# Autodesk Inventor assembly: Arm_v2
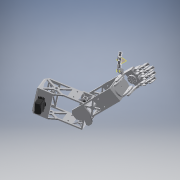
[picture p0: Inventor's stored thumbnail of the model, 180x180]
Saved by Autodesk Inventor 2018 (Build 220112000, 112)
## iProperties
Created: 2018-04-13
Part Number: Arm_v2
Material: Générique
Document SubType Name: Assembly
Designer: Thomas
Author: Thomas
## Documents named in this file (7)
- D:\Users\Thomas\Desktop\Projet robot augmenté\armConcept_v1\Robot simplifié\Arm_v2.iam
- D:\Users\Thomas\Desktop\Projet robot augmenté\armConcept_v1\Robot simplifié\Biceps1 v2.ipt
- D:\Users\Thomas\Desktop\Projet robot augmenté\armConcept_v1\Robot simplifié\Biceps2 v2.ipt
- D:\Users\Thomas\Desktop\Projet robot augmenté\armConcept_v1\MG996R SERVO\MG_996R.iam
- D:\Users\Thomas\Desktop\Projet robot augmenté\armConcept_v1\Robot simplifié\Forearm1 v2.ipt
- D:\Users\Thomas\Desktop\Projet robot augmenté\armConcept_v1\Robot simplifié\Forearm2 v2.ipt
- D:\Users\Thomas\Desktop\Projet robot augmenté\armConcept_v1\Hand\Full hand.iam
## Components (7 placed, 6 different names)
1. Biceps1 v2:1 — Placage:1, Placage:2, Placage:3, Placage:6, Rotation:1
2. Biceps2 v2:1 — Placage:1, Placage:2, Placage:3, Rotation:2, Rotation:3
3. MG_996R:1 [sub-assembly] — Rotation:2, Rotation:3, Rotation:4
4. MG_996R:2 [sub-assembly] — Placage:6, Rotation:1
5. Forearm1 v2:1 — Rotation:4, Placage:7, Placage:8, Placage:9
6. Forearm2 v2:1 — Placage:7, Placage:8, Placage:9, Rotation:5
7. Full hand:1 [sub-assembly] — Rotation:5
## Relationships (12: Mate 7, RevoluteJoint 5)
- Placage:1 [Mate]: Biceps1 v2:1 ↔ Biceps2 v2:1
- Placage:2 [Mate]: Biceps1 v2:1 ↔ Biceps2 v2:1
- Placage:3 [Mate]: Biceps1 v2:1 ↔ Biceps2 v2:1
- Placage:6 [Mate]: Biceps1 v2:1 ↔ MG_996R:2
- Rotation:1 [RevoluteJoint]: Biceps1 v2:1 ↔ MG_996R:2
- Rotation:2 [RevoluteJoint]: Biceps2 v2:1 ↔ MG_996R:1
- Rotation:3 [RevoluteJoint]: Biceps2 v2:1 ↔ MG_996R:1
- Rotation:4 [RevoluteJoint]: MG_996R:1 ↔ Forearm1 v2:1
- Placage:7 [Mate]: Forearm1 v2:1 ↔ Forearm2 v2:1
- Placage:8 [Mate]: Forearm1 v2:1 ↔ Forearm2 v2:1
- Placage:9 [Mate]: Forearm1 v2:1 ↔ Forearm2 v2:1
- Rotation:5 [RevoluteJoint]: Forearm2 v2:1 ↔ Full hand:1
